# Autodesk Inventor assembly: EL1-100
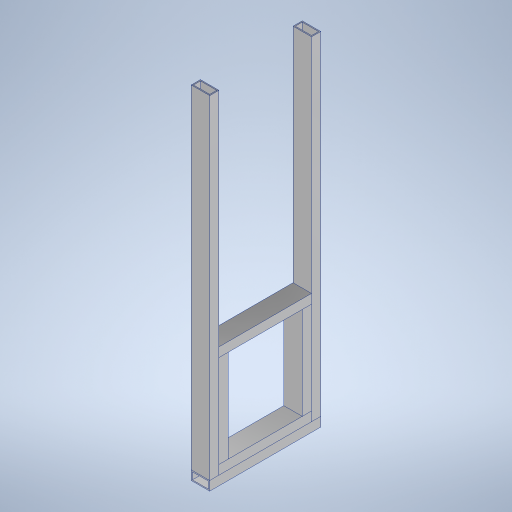
[picture p0: Inventor's stored thumbnail of the model, 512x512]
Saved by Autodesk Inventor 2023.4 (Build 274418000, 418)
## iProperties
Created: 2025-01-09
Part Number: EL1-100
Document SubType Name: Assembly
Designer: mavericks
Author: mavericks
## Documents named in this file (4)
- C:\Users\mavericks\Desktop\2025-ReefScape---CAD\Elevator\EL1-100.iam
- C:\Users\mavericks\Desktop\2025-ReefScape---CAD\Elevator\EL1-001.ipt
- C:\Users\mavericks\Desktop\2025-ReefScape---CAD\Elevator\EL1-002.ipt
- C:\Users\mavericks\Desktop\2025-ReefScape---CAD\Elevator\EL1-003.ipt
## Components (7 placed, 3 different names)
1. EL1-002:1 — Mate:1, Flush:1, Flush:2
2. EL1-002:2 — Flush:3, Flush:4, Mate:2, Flush:11, Mate:6
3. EL1-001:1 — Mate:1, Flush:1, Flush:2, Flush:3, Flush:4, Mate:2, Mate:7
4. EL1-003:1 — Mate:5, Flush:9, Flush:10, Flush:11
5. EL1-003:2 — Mate:3, Flush:5, Flush:6, Flush:7, Flush:8, Mate:4, Mate:7
6. EL1-003:3 — Mate:3, Flush:5, Flush:6, Flush:9, Flush:10, Mate:6
7. EL1-003:4 — Flush:7, Flush:8, Mate:4, Mate:5
## Relationships (18: Flush 11, Mate 7)
- Mate:1: EL1-002:1 ↔ EL1-001:1
- Flush:1: EL1-002:1 ↔ EL1-001:1
- Flush:2: EL1-002:1 ↔ EL1-001:1
- Flush:3: EL1-002:2 ↔ EL1-001:1
- Flush:4: EL1-002:2 ↔ EL1-001:1
- Mate:2: EL1-002:2 ↔ EL1-001:1
- Mate:3: EL1-003:2 ↔ EL1-003:3
- Flush:5: EL1-003:2 ↔ EL1-003:3
- Flush:6: EL1-003:2 ↔ EL1-003:3
- Flush:7: EL1-003:2 ↔ EL1-003:4
- Flush:8: EL1-003:2 ↔ EL1-003:4
- Mate:4: EL1-003:2 ↔ EL1-003:4
- Mate:5: EL1-003:1 ↔ EL1-003:4
- Flush:9: EL1-003:1 ↔ EL1-003:3
- Flush:10: EL1-003:1 ↔ EL1-003:3
- Flush:11: EL1-002:2 ↔ EL1-003:1
- Mate:6: EL1-002:2 ↔ EL1-003:3
- Mate:7: EL1-001:1 ↔ EL1-003:2
